# Autodesk Inventor assembly: Housing 4
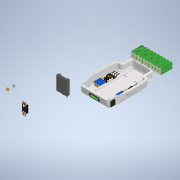
[picture p0: Inventor's stored thumbnail of the model, 180x180]
Saved by Autodesk Inventor 2020.1 (Build 241239000, 239)
## iProperties
Created: 2019-11-16
Part Number: Housing 4
Document SubType Name: Assembly
Designer: Petar
Author: Petar
## Documents named in this file (9)
- D:\OMG\E-Board\CAD\Inventor\Housing\Housing 4.iam
- D:\OMG\E-Board\CAD\Inventor\Housing\Battery Housing Box v3.ipt
- D:\OMG\E-Board\CAD\Inventor\Electrical Components\Battery Indicator.ipt
- D:\OMG\E-Board\CAD\Inventor\Electrical Components\BMS (separate port).ipt
- D:\OMG\E-Board\CAD\Inventor\Electrical Components\Battery Pack\Samsung 25R\Battery Pack - Samsung 25R - 2xRows.iam
- D:\OMG\E-Board\CAD\Inventor\Electrical Components\Power Switch - detail.ipt
- D:\OMG\E-Board\CAD\Inventor\Electrical Components\Power Button.ipt
- D:\OMG\E-Board\CAD\Inventor\Electrical Components\VESC - detail.ipt
- D:\OMG\E-Board\CAD\Inventor\Electrical Components\XLR Female Plug.ipt
## Components (9 placed, 8 different names)
1. Battery Housing Box v3:1 — Rotational:1, Rotational:2, Rigid:1, Rigid:2
2. Battery Indicator:1 — Rotational:1
3. BMS (separate port):1
4. Battery Pack - Samsung 25R - 2xRows:1 [sub-assembly]
5. Power Switch - detail:1
6. Power Button:1
7. VESC - detail:1 — Rigid:1
8. VESC - detail:2 — Rigid:2
9. XLR Female Plug:1 — Rotational:2
## Relationships (4: RevoluteJoint 2, WeldJoint 2)
- Rotational:1 [RevoluteJoint]: Battery Housing Box v3:1 ↔ Battery Indicator:1
- Rotational:2 [RevoluteJoint]: Battery Housing Box v3:1 ↔ XLR Female Plug:1
- Rigid:1 [WeldJoint] (7 mm): Battery Housing Box v3:1 ↔ VESC - detail:1
- Rigid:2 [WeldJoint] (7 mm): Battery Housing Box v3:1 ↔ VESC - detail:2
